# Autodesk Inventor assembly: Assembly
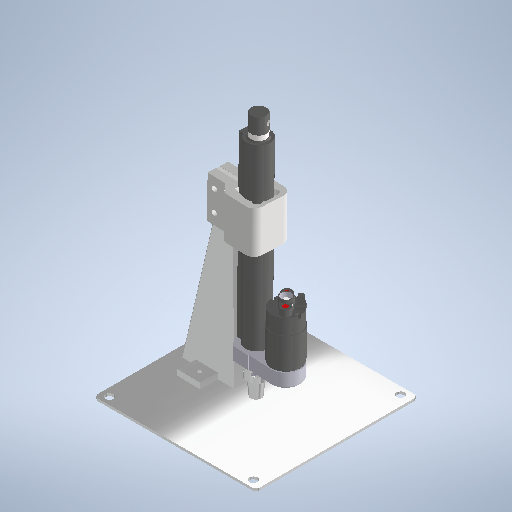
[picture p0: Inventor's stored thumbnail of the model, 512x512]
Saved by Autodesk Inventor 2025.3 (Build 293356000, 356)
## iProperties
Created: 2025-10-10
Part Number: Assembly
Document SubType Name: Assembly
Designer: Haggag
Author: Haggag
## Documents named in this file (7)
- C:\Users\Haggag\Documents\Lifting Mechanism\Assembly.iam
- C:\Users\Haggag\Documents\Lifting Mechanism\Base.ipt
- C:\Users\Haggag\Documents\Lifting Mechanism\LinearActuator\LinearActuator.iam
- C:\Users\Haggag\Documents\Lifting Mechanism\Linear Actuator Base Holder.ipt
- C:\Users\Haggag\Documents\Lifting Mechanism\Bracket.ipt
- C:\Users\Haggag\Documents\Inventor\Content Center Files\R2025\en-US\ISO 7046-1 H(1)\ISO 7046-1 - M5 x 16_ - 4.8 - H - ISO.ipt
- C:\Users\Haggag\Documents\Lifting Mechanism\Spine.ipt
## Components (6 placed, 6 different names)
1. Base:1 — Mate:1, Rotational:1
2. LinearActuator:1 [sub-assembly] — Cylindrical:2, Cylindrical:3
3. Linear Actuator Base Holder:1 — Cylindrical:2, Mate:1
4. Bracket:1 — Cylindrical:3, Rotational:2, Mate:2
5. ISO 7046-1 H M5 x 16 - 4.8 - H:1 — Rotational:1
6. Spine:1 — Rotational:2, Mate:2
## Relationships (6: CylindricalJoint 2, Mate 2, RevoluteJoint 2)
- Cylindrical:2: LinearActuator:1 ↔ Linear Actuator Base Holder:1
- Mate:1: Base:1 ↔ Linear Actuator Base Holder:1
- Cylindrical:3: LinearActuator:1 ↔ Bracket:1
- Rotational:1 [RevoluteJoint]: Base:1 ↔ ISO 7046-1 H M5 x 16 - 4.8 - H:1
- Rotational:2 [RevoluteJoint]: Bracket:1 ↔ Spine:1
- Mate:2: Bracket:1 ↔ Spine:1
